# Autodesk Inventor assembly: sail_hold_assembly
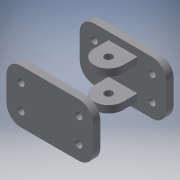
[picture p0: Inventor's stored thumbnail of the model, 180x180]
Saved by Autodesk Inventor 2016 (Build 200138000, 138)
## iProperties
Created: 2015-09-21
Part Number: sail_hold_assembly
Document SubType Name: Assembly
Designer: Qiuyang
Author: Qiuyang
## Documents named in this file (3)
- C:\Users\Qiuyang\Dropbox\Senior_Design\SailBoat\Document\sail_hold_assembly.iam
- C:\Users\Qiuyang\Dropbox\Senior_Design\SailBoat\Document\sail_hold_1.ipt
- C:\Users\Qiuyang\Dropbox\Senior_Design\SailBoat\Document\sail_hold_2.ipt
## Components (2 placed, 2 different names)
1. sail_hold_1:1 — Insert:1
2. sail_hold_2:1 — Insert:1
## Relationships (1: Insert 1)
- Insert:1 (50.8 mm): sail_hold_1:1 ↔ sail_hold_2:1
